# Autodesk Inventor assembly: Thermal cover assembly
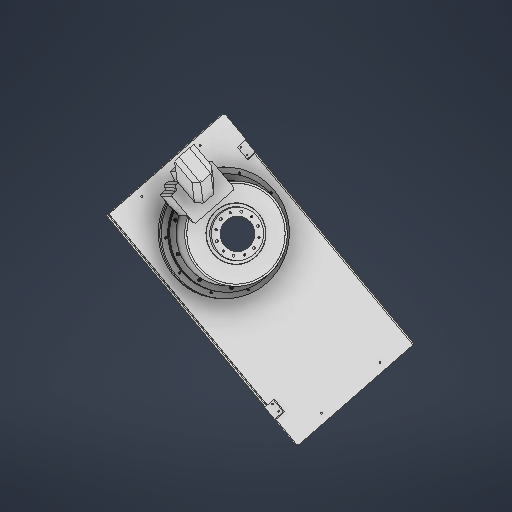
[picture p0: Inventor's stored thumbnail of the model, 512x512]
Saved by Autodesk Inventor 2025 (Build 290162000, 162)
## iProperties
Created: 2025-07-25
Part Number: Thermal cover assembly
Document SubType Name: Assembly
Designer: mateo
Author: mateo
## Documents named in this file (14)
- C:\Users\mayhe\OneDrive\Documents\GitHub\In-situ-monitoring-of-powder-bed-fusion-additive-manufacturing\system_development\Adamant\v0.1\hardware design\Thermal cover assembly.iam
- C:\Users\mayhe\OneDrive\Documents\GitHub\In-situ-monitoring-of-powder-bed-fusion-additive-manufacturing\system_development\Adamant\v0.1\hardware design\Cover (Thermal Camera).ipt
- C:\Users\mayhe\OneDrive\Documents\GitHub\In-situ-monitoring-of-powder-bed-fusion-additive-manufacturing\system_development\Adamant\v0.1\hardware design\300mm Housing 1.ipt
- C:\Users\mayhe\OneDrive\Documents\GitHub\In-situ-monitoring-of-powder-bed-fusion-additive-manufacturing\system_development\Adamant\v0.1\hardware design\300mm housing 2 Camera.ipt
- C:\Users\mayhe\OneDrive\Documents\GitHub\In-situ-monitoring-of-powder-bed-fusion-additive-manufacturing\system_development\Adamant\v0.1\hardware design\Cylinder Segment  Camera only v0.2.ipt
- C:\Users\mayhe\OneDrive\Documents\GitHub\In-situ-monitoring-of-powder-bed-fusion-additive-manufacturing\system_development\Adamant\v0.1\hardware design\Cylinder Slidey Bit Housing Camera only v0.2.ipt
- C:\Users\mayhe\OneDrive\Documents\GitHub\In-situ-monitoring-of-powder-bed-fusion-additive-manufacturing\system_development\Adamant\v0.1\hardware design\Cylinder Segment Holder.ipt
- C:\Users\mayhe\OneDrive\Documents\GitHub\In-situ-monitoring-of-powder-bed-fusion-additive-manufacturing\system_development\Adamant\v0.1\hardware design\Cylinder Segment Camera Only\C .Replace - 10.ipt
- C:\GitHub\In-situ-monitoring-of-powder-bed-fusion-additive-manufacturing\system_development\Adamant\v0.1\hardware design\Cylinder Segment Camera Only.ipt
- C:\Users\mayhe\OneDrive\Documents\GitHub\In-situ-monitoring-of-powder-bed-fusion-additive-manufacturing\system_development\Adamant\v0.1\hardware design\Thermal Camera Bracket.ipt
- C:\Users\mayhe\OneDrive\Documents\GitHub\In-situ-monitoring-of-powder-bed-fusion-additive-manufacturing\system_development\Adamant\v0.1\hardware design\C .Replace - Face.ipt
- C:\Users\mayhe\OneDrive\Documents\GitHub\In-situ-monitoring-of-powder-bed-fusion-additive-manufacturing\system_development\Adamant\v0.1\hardware design\Thermal Cover.ipt
- C:\Users\mayhe\OneDrive\Documents\GitHub\In-situ-monitoring-of-powder-bed-fusion-additive-manufacturing\system_development\Adamant\v0.1\hardware design\Welding Glass.ipt
- C:\Users\mayhe\OneDrive\Documents\GitHub\In-situ-monitoring-of-powder-bed-fusion-additive-manufacturing\system_development\Adamant\v0.1\hardware design\Xi-410-Camera-with-29°-x-18°-Lens\Xi 410 Camera with 29° x.iam
## Components (12 placed, 12 different names)
1. Cover (Thermal Camera):1 — Insert:1, Insert:2, Insert:3
2. 300mm Housing 1:1 — Insert:1, Insert:2, Insert:3, Insert:4, Insert:5
3. 300mm housing 2 Camera:1 — Insert:4, Insert:5, Insert:6, Insert:7
4. Cylinder Segment  Camera only v0.2:1 — Insert:6, Insert:7, Insert:8, Insert:9, Insert:10, Insert:11, Rotational:2, Mate:4
5. Cylinder Slidey Bit Housing Camera only v0.2:1 — Insert:8, Insert:9, Insert:14, Insert:15, Mate:2
6. Cylinder Segment Holder:1 — Insert:10, Insert:11, Insert:12, Insert:13
7. C .Replace - 10:1 — Insert:12
8. Thermal Camera Bracket:1 — Insert:14, Insert:15, Rotational:1, Mate:3
9. C .Replace - Face:2 — Insert:13
10. Thermal Cover:1 — Rotational:2, Mate:4
11. Welding Glass:1 — Mate:2
12. Xi 410 Camera with 29° x:1 [sub-assembly] — Rotational:1, Mate:3
## Relationships (20: Insert 15, Mate 3, RevoluteJoint 2)
- Insert:1: Cover (Thermal Camera):1 ↔ 300mm Housing 1:1
- Insert:2: Cover (Thermal Camera):1 ↔ 300mm Housing 1:1
- Insert:3: Cover (Thermal Camera):1 ↔ 300mm Housing 1:1
- Insert:4: 300mm Housing 1:1 ↔ 300mm housing 2 Camera:1
- Insert:5: 300mm Housing 1:1 ↔ 300mm housing 2 Camera:1
- Insert:6 (10 mm): 300mm housing 2 Camera:1 ↔ Cylinder Segment  Camera only v0.2:1
- Insert:7 (10 mm): 300mm housing 2 Camera:1 ↔ Cylinder Segment  Camera only v0.2:1
- Insert:8: Cylinder Segment  Camera only v0.2:1 ↔ Cylinder Slidey Bit Housing Camera only v0.2:1
- Insert:9: Cylinder Segment  Camera only v0.2:1 ↔ Cylinder Slidey Bit Housing Camera only v0.2:1
- Insert:10: Cylinder Segment  Camera only v0.2:1 ↔ Cylinder Segment Holder:1
- Insert:11: Cylinder Segment  Camera only v0.2:1 ↔ Cylinder Segment Holder:1
- Insert:12: Cylinder Segment Holder:1 ↔ C .Replace - 10:1
- Insert:13: Cylinder Segment Holder:1 ↔ C .Replace - Face:2
- Insert:14: Cylinder Slidey Bit Housing Camera only v0.2:1 ↔ Thermal Camera Bracket:1
- Insert:15: Cylinder Slidey Bit Housing Camera only v0.2:1 ↔ Thermal Camera Bracket:1
- Mate:2: Cylinder Slidey Bit Housing Camera only v0.2:1 ↔ Welding Glass:1
- Rotational:1 [RevoluteJoint]: Thermal Camera Bracket:1 ↔ Xi 410 Camera with 29° x:1
- Mate:3: Thermal Camera Bracket:1 ↔ Xi 410 Camera with 29° x:1
- Rotational:2 [RevoluteJoint]: Cylinder Segment  Camera only v0.2:1 ↔ Thermal Cover:1
- Mate:4: Cylinder Segment  Camera only v0.2:1 ↔ Thermal Cover:1
